# Autodesk Inventor assembly: reductor_12_10_ass
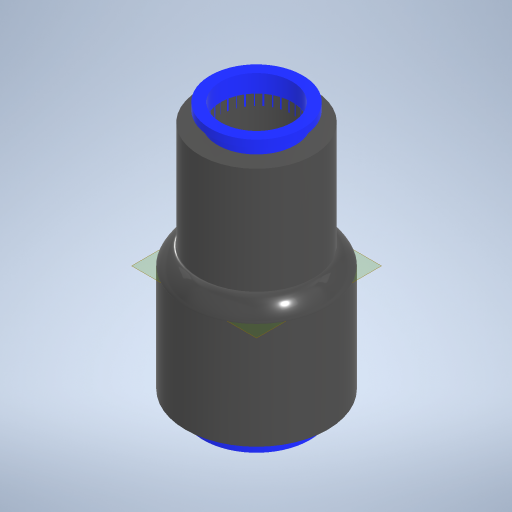
[picture p0: Inventor's stored thumbnail of the model, 512x512]
Saved by Autodesk Inventor 2024 (Build 280153000, 153)
## iProperties
Created: 2023-04-11
Part Number: reductor_12_10_ass
Document SubType Name: Assembly
Designer: ferna
Author: ferna
## Documents named in this file (4)
- C:\Users\ferna\OneDrive - Universidad Católica de Chile\Bocas\RobotFlautista\reductor_12_10_ass.iam
- C:\Users\ferna\OneDrive - Universidad Católica de Chile\Bocas\RobotFlautista\reductor1210.ipt
- C:\Users\ferna\OneDrive - Universidad Católica de Chile\Bocas\RobotFlautista\entrada_manguera_2.ipt
- C:\Users\ferna\OneDrive - Universidad Católica de Chile\Bocas\RobotFlautista\entrada_manguera_2_big.ipt
## Components (3 placed, 3 different names)
1. reductor1210:1 — Mate:1, Mate:2, Mate:3, Mate:4
2. entrada_manguera_2:1 — Mate:3, Mate:4
3. entrada_manguera_2_big:1 — Mate:1, Mate:2
## Relationships (4: Mate 4)
- Mate:1 (-1.5 mm): reductor1210:1 ↔ entrada_manguera_2_big:1
- Mate:2: reductor1210:1 ↔ entrada_manguera_2_big:1
- Mate:3 (-1.5 mm): reductor1210:1 ↔ entrada_manguera_2:1
- Mate:4: reductor1210:1 ↔ entrada_manguera_2:1
